# Autodesk Inventor assembly: right_part
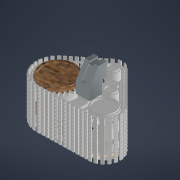
[picture p0: Inventor's stored thumbnail of the model, 180x180]
Saved by Autodesk Inventor 2022 (Build 260153000, 153)
## iProperties
Created: 2021-12-31
Part Number: right_part
Document SubType Name: Assembly
Designer: MatusBarany
Author: MatusBarany
## Documents named in this file (12)
- C:\Users\Public\Documents\Autodesk\Inventor 2022\Projects\wall-e\right_part.iam
- C:\Users\Public\Documents\Autodesk\Inventor 2022\Projects\wall-e\wheel connector.ipt
- C:\Users\Public\Documents\Autodesk\Inventor 2022\Projects\wall-e\under walle L3.ipt
- C:\Users\Public\Documents\Autodesk\Inventor 2022\Projects\wall-e\uchytka_spojky_medzi_velkym_strednym.ipt
- C:\Users\Public\Documents\Autodesk\Inventor 2022\Projects\wall-e\spojka_pol_velke_koleso.ipt
- C:\Users\Public\Documents\Autodesk\Inventor 2022\Projects\wall-e\spojka_pol_stredne_koleso.ipt
- C:\Users\Public\Documents\Autodesk\Inventor 2022\Projects\wall-e\velke_koleso.ipt
- C:\Users\Public\Documents\Autodesk\Inventor 2022\Projects\wall-e\stredne_koleso.ipt
- C:\Users\Public\Documents\Autodesk\Inventor 2022\Projects\wall-e\male_koliesko.ipt
- C:\Users\Public\Documents\Autodesk\Inventor 2022\Projects\wall-e\spojka_male_koleso.ipt
- C:\Users\Public\Documents\Autodesk\Inventor 2022\Projects\wall-e\onePart_chain.ipt
- C:\Users\Public\Documents\Autodesk\Inventor 2022\Projects\wall-e\chain right.ipt
## Components (68 placed, 11 different names)
1. wheel connector:1 — Mate:1, Mate:2, Mate:3, Mate:4, Mate:5, Mate:6, Rotational:1
2. under walle L3:1 — Mate:1, Mate:2, Mate:3
3. uchytka_spojky_medzi_velkym_strednym:1 — Mate:4, Mate:5, Mate:6, Mate:7, Cylindrical:1
4. spojka_pol_velke_koleso:1 — Mate:7, Cylindrical:1, Mate:8, Flush:1, Flush:2, Rigid:1, Rigid:2
5. spojka_pol_stredne_koleso:1 — Mate:8, Flush:1, Flush:2, Rigid:3, Rigid:4
6. velke_koleso:1 — Rigid:1, Flush:3
7. velke_koleso:2 — Rigid:2
8. stredne_koleso:1 — Rigid:3
9. stredne_koleso:2 — Rigid:4
10. male_koliesko:1 — Rigid:6
11. male_koliesko:2 — Rigid:9
12. male_koliesko:3 — Rigid:8
13. male_koliesko:4 — Rigid:7
14. spojka_male_koleso:1 — Rigid:6, Rigid:7, Rigid:8, Rigid:9, Rotational:1
15. chain right:1 — Flush:4, Flush:5, Flush:6, Mate:9, Mate:10
16. onePart_chain:1 — Flush:6, Mate:9, Mate:10
17. onePart_chain:2
18. onePart_chain:3
19. onePart_chain:4
20. onePart_chain:5
21. onePart_chain:6
22. onePart_chain:7
23. onePart_chain:8
24. onePart_chain:9
25. onePart_chain:10
26. onePart_chain:11
27. onePart_chain:12
28. onePart_chain:13
29. onePart_chain:14
30. onePart_chain:15
31. onePart_chain:16
32. onePart_chain:17
33. onePart_chain:18
34. onePart_chain:19
35. onePart_chain:20
36. onePart_chain:21
37. onePart_chain:22
38. onePart_chain:23
39. onePart_chain:24
40. onePart_chain:25
41. onePart_chain:26
42. onePart_chain:27
43. onePart_chain:28
44. onePart_chain:29
45. onePart_chain:30
46. onePart_chain:31
47. onePart_chain:32
48. onePart_chain:33
49. onePart_chain:34
50. onePart_chain:35
51. onePart_chain:36
52. onePart_chain:37
53. onePart_chain:38
54. onePart_chain:39
55. onePart_chain:40
56. onePart_chain:41
57. onePart_chain:42
58. onePart_chain:43
59. onePart_chain:44
60. onePart_chain:45
61. onePart_chain:46
62. onePart_chain:47
63. onePart_chain:48
64. onePart_chain:49
65. onePart_chain:50
66. onePart_chain:51
67. onePart_chain:52
68. onePart_chain:53
## Component patterns: (53 elements, first: onePart_chain:1)
## Relationships (26: Mate 10, WeldJoint 8, Flush 6, CylindricalJoint 1, RevoluteJoint 1)
- Mate:1: wheel connector:1 ↔ under walle L3:1
- Mate:2: wheel connector:1 ↔ under walle L3:1
- Mate:3: wheel connector:1 ↔ under walle L3:1
- Mate:4: wheel connector:1 ↔ uchytka_spojky_medzi_velkym_strednym:1
- Mate:5: wheel connector:1 ↔ uchytka_spojky_medzi_velkym_strednym:1
- Mate:6: wheel connector:1 ↔ uchytka_spojky_medzi_velkym_strednym:1
- Mate:7: uchytka_spojky_medzi_velkym_strednym:1 ↔ spojka_pol_velke_koleso:1
- Cylindrical:1: uchytka_spojky_medzi_velkym_strednym:1 ↔ spojka_pol_velke_koleso:1
- Mate:8: spojka_pol_velke_koleso:1 ↔ spojka_pol_stredne_koleso:1
- Flush:1: spojka_pol_velke_koleso:1 ↔ spojka_pol_stredne_koleso:1
- Flush:2: spojka_pol_velke_koleso:1 ↔ spojka_pol_stredne_koleso:1
- Rigid:1 [WeldJoint]: spojka_pol_velke_koleso:1 ↔ velke_koleso:1
- Rigid:2 [WeldJoint]: spojka_pol_velke_koleso:1 ↔ velke_koleso:2
- Rigid:3 [WeldJoint]: spojka_pol_stredne_koleso:1 ↔ stredne_koleso:1
- Rigid:4 [WeldJoint]: spojka_pol_stredne_koleso:1 ↔ stredne_koleso:2
- Rigid:6 [WeldJoint]: male_koliesko:1 ↔ spojka_male_koleso:1
- Rigid:7 [WeldJoint]: male_koliesko:4 ↔ spojka_male_koleso:1
- Rigid:8 [WeldJoint]: male_koliesko:3 ↔ spojka_male_koleso:1
- Rigid:9 [WeldJoint]: male_koliesko:2 ↔ spojka_male_koleso:1
- Flush:3 (-1.5 mm): velke_koleso:1
- Flush:4: chain right:1
- Flush:5: chain right:1
- Flush:6: chain right:1 ↔ onePart_chain:1
- Mate:9: chain right:1 ↔ onePart_chain:1
- Mate:10: chain right:1 ↔ onePart_chain:1
- Rotational:1 [RevoluteJoint]: wheel connector:1 ↔ spojka_male_koleso:1
